# Autodesk Inventor assembly: s-assy-scara-unit-j2_sub
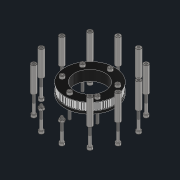
[picture p0: Inventor's stored thumbnail of the model, 180x180]
Saved by Autodesk Inventor 2022 (Build 260153000, 153)
## iProperties
Created: 2021-07-12
Document SubType Name: Assembly
Designer: yuta0
Mass: 2750.98 g
Surface Area: 6960.57 cm^2
Volume: 1238.47 cm^3
Density: 2.22127 g/cm^3
Part Number: s-assy-scara-unit-j2_sub
Author: yuta0
## Documents named in this file (6)
- C:\Users\yuta0\Desktop\assy-scara\s-assy-scara-unit-j2_sub.iam
- C:\Users\yuta0\Desktop\assy-scara\scara-base2.ipt
- C:\Users\yuta0\Desktop\assy-scara\CB4-35.ipt
- C:\Users\yuta0\Desktop\assy-scara\ARF-440E.ipt
- C:\Users\yuta0\Desktop\assy-scara\LBNR4.ipt
- C:\Users\yuta0\Documents\GitHub\catchrobo_hardware\assy-robot\s-assy-unit-j3.iam
## Components (31 placed, 4 different names)
1. scara-base2:1 — メイト:113, メイト:114
2. CB4-35:2 — メイト:113, メイト:114
3. CB4-35:3
4. CB4-35:4
5. CB4-35:5
6. CB4-35:6
7. CB4-35:7
8. ARF-440E:1
9. CB4-35:8
10. ARF-440E:2
11. CB4-35:9
12. ARF-440E:3
13. CB4-35:10
14. ARF-440E:4
15. CB4-35:11
16. ARF-440E:5
17. CB4-35:12
18. ARF-440E:6
19. CB4-35:13
20. ARF-440E:7
21. CB4-35:14
22. ARF-440E:8
23. CB4-35:15
24. ARF-440E:9
25. CB4-35:16
26. ARF-440E:10
27. CB4-35:17
28. CB4-35:18 — メイト:121
29. LBNR4:1 — メイト:121
30. CB4-35:19
31. LBNR4:2
## Component patterns: (6 elements, first: CB4-35:2), (10 elements, first: ARF-440E:1 + CB4-35:8), (2 elements, first: CB4-35:18 + LBNR4:1)
## Relationships (3: Mate 3)
- メイト:113 [Mate]: scara-base2:1 ↔ CB4-35:2
- メイト:114 [Mate]: scara-base2:1 ↔ CB4-35:2
- メイト:121 [Mate]: CB4-35:18 ↔ LBNR4:1
